# Autodesk Inventor assembly: GoPro Hero 3 HD Camera
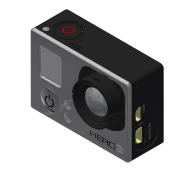
[picture p0: Inventor's stored thumbnail of the model, 180x180]
Saved by Autodesk Inventor 2015 (Build 190159000, 159)
## iProperties
Created: 2013-02-14
Document SubType Name: Assembly
Designer: sdarley
Project: GoPro Hero 3 HD Camera
Description: GoPro Hero 3 HD Camera
Vendor: GoPro
Stock Number: Hero 3
Author: sdarley
Title: GoPro Hero 3 HD Camera
Revision Number: 1
## Documents named in this file (10)
- C:\Users\Antonella\Documents\Inventor\SphereCam\GoPro Hero 3 HD Camera\GoPro Hero 3 HD Camera.iam
- C:\Users\Antonella\Documents\Inventor\SphereCam\GoPro Hero 3 HD Camera\GoPro Hero 3 Front Panel.ipt
- C:\Users\Antonella\Documents\Inventor\SphereCam\GoPro Hero 3 HD Camera\GoPro Hero 3 Screen.ipt
- C:\Users\Antonella\Documents\Inventor\SphereCam\GoPro Hero 3 HD Camera\GoPro Hero 3 Mode Button.ipt
- C:\Users\Antonella\Documents\Inventor\SphereCam\GoPro Hero 3 HD Camera\GoPro Hero 3 LED Cover.ipt
- C:\Users\Antonella\Documents\Inventor\SphereCam\GoPro Hero 3 HD Camera\GoPro Hero 3 Housing.ipt
- C:\Users\Antonella\Documents\Inventor\SphereCam\GoPro Hero 3 HD Camera\GoPro Hero 3 Lens.ipt
- C:\Users\Antonella\Documents\Inventor\SphereCam\GoPro Hero 3 HD Camera\micro sd.iam
- C:\Users\Antonella\Documents\Inventor\SphereCam\GoPro Hero 3 HD Camera\GoPro Hero 3 Indicator Cover.ipt
- C:\Users\Antonella\Documents\Inventor\SphereCam\GoPro Hero 3 HD Camera\GoPro Hero 3 HDMI pin.ipt
## Components (20 placed, 9 different names)
1. GoPro Hero 3 Front Panel:1 — Flush:1, Mate:1, Mate:2, Flush:2, Insert:1, Mate:3, Flush:3, Insert:2, Insert:3, Flush:4, Mate:4, Flush:5
2. GoPro Hero 3 Screen:1 — Flush:1, Mate:1, Mate:2
3. GoPro Hero 3 Mode Button:1 — Flush:2, Insert:1, Mate:3
4. GoPro Hero 3 LED Cover:1 — Flush:3, Insert:2
5. GoPro Hero 3 LED Cover:2 — Insert:3
6. GoPro Hero 3 Housing:1 — Flush:4, Insert:4, Mate:4, Flush:5, Flush:6, Flush:7, Mate:5, Insert:5, Insert:6, Insert:7, Flush:8, Mate:6, Mate:7
7. GoPro Hero 3 Lens:1 — Insert:4
8. GoPro Hero 3 Indicator Cover:1 — Insert:5
9. GoPro Hero 3 Indicator Cover:2 — Insert:6
10. GoPro Hero 3 Indicator Cover:3 — Insert:7
11. micro sd:1 [sub-assembly] — Flush:6, Flush:7, Mate:5
12. GoPro Hero 3 HDMI pin:1 — Flush:8, Mate:6, Mate:7
13. GoPro Hero 3 HDMI pin:2
14. GoPro Hero 3 HDMI pin:3
15. GoPro Hero 3 HDMI pin:4
16. GoPro Hero 3 HDMI pin:5
17. GoPro Hero 3 HDMI pin:6
18. GoPro Hero 3 HDMI pin:7
19. GoPro Hero 3 HDMI pin:8
20. GoPro Hero 3 HDMI pin:9
## Component patterns: (9 elements, first: GoPro Hero 3 HDMI pin:1)
## Relationships (22: Flush 8, Mate 7, Insert 7)
- Flush:1: GoPro Hero 3 Front Panel:1 ↔ GoPro Hero 3 Screen:1
- Mate:1 (5 mm): GoPro Hero 3 Front Panel:1 ↔ GoPro Hero 3 Screen:1
- Mate:2 (4 mm): GoPro Hero 3 Front Panel:1 ↔ GoPro Hero 3 Screen:1
- Flush:2: GoPro Hero 3 Front Panel:1 ↔ GoPro Hero 3 Mode Button:1
- Insert:1: GoPro Hero 3 Front Panel:1 ↔ GoPro Hero 3 Mode Button:1
- Mate:3: GoPro Hero 3 Front Panel:1 ↔ GoPro Hero 3 Mode Button:1
- Flush:3: GoPro Hero 3 Front Panel:1 ↔ GoPro Hero 3 LED Cover:1
- Insert:2: GoPro Hero 3 Front Panel:1 ↔ GoPro Hero 3 LED Cover:1
- Insert:3: GoPro Hero 3 Front Panel:1 ↔ GoPro Hero 3 LED Cover:2
- Flush:4: GoPro Hero 3 Front Panel:1 ↔ GoPro Hero 3 Housing:1
- Insert:4: GoPro Hero 3 Housing:1 ↔ GoPro Hero 3 Lens:1
- Mate:4: GoPro Hero 3 Front Panel:1 ↔ GoPro Hero 3 Housing:1
- Flush:5: GoPro Hero 3 Front Panel:1 ↔ GoPro Hero 3 Housing:1
- Flush:6 (-2 mm): GoPro Hero 3 Housing:1 ↔ micro sd:1
- Flush:7 (-0.5 mm): GoPro Hero 3 Housing:1 ↔ micro sd:1
- Mate:5 (0.2 mm): GoPro Hero 3 Housing:1 ↔ micro sd:1
- Insert:5: GoPro Hero 3 Housing:1 ↔ GoPro Hero 3 Indicator Cover:1
- Insert:6: GoPro Hero 3 Housing:1 ↔ GoPro Hero 3 Indicator Cover:2
- Insert:7: GoPro Hero 3 Housing:1 ↔ GoPro Hero 3 Indicator Cover:3
- Flush:8: GoPro Hero 3 Housing:1 ↔ GoPro Hero 3 HDMI pin:1
- Mate:6: GoPro Hero 3 Housing:1 ↔ GoPro Hero 3 HDMI pin:1
- Mate:7: GoPro Hero 3 Housing:1 ↔ GoPro Hero 3 HDMI pin:1
